# Autodesk Inventor assembly: Antriebsstrang
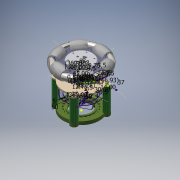
[picture p0: Inventor's stored thumbnail of the model, 180x180]
Saved by Autodesk Inventor 2018.3 (Build 223284000, 284)
## iProperties
Created: 2018-06-25
Part Number: Antriebsstrang
Material: Generisch
Document SubType Name: Assembly
Designer: JochenAlt
Author: JochenAlt
## Documents named in this file (5)
- D:\Projects\FlowerPot\CAD\Antriebsstrang.iam
- D:\Projects\FlowerPot\CAD\OmniWheel.ipt
- D:\Projects\FlowerPot\CAD\HarmonicDrive.iam
- D:\Projects\FlowerPot\CAD\Mounting Hub.ipt
- C:\Users\JochenAlt\Documents\Inventor\Content Center Files\R2018\de-DE\SKF - Single row ball bearings\SKF604.ipt
## Components (4 placed, 4 different names)
1. OmniWheel:1 — Passend:1, Passend:6, Passend:7, Passend:8
2. HarmonicDrive:1 [sub-assembly] — Passend:2, Passend:4, Passend:5, Passend:6
3. Mounting Hub:1 — Passend:1, Passend:2, Passend:5, Passend:7, Passend:8, Passend:9
4. SKF- Kugellager, einreihig SKF604:1 — Passend:4, Passend:9
## Relationships (8: Mate 8)
- Passend:1 [Mate]: OmniWheel:1 ↔ Mounting Hub:1
- Passend:2 [Mate]: HarmonicDrive:1 ↔ Mounting Hub:1
- Passend:4 [Mate]: HarmonicDrive:1 ↔ SKF- Kugellager, einreihig SKF604:1
- Passend:5 [Mate]: HarmonicDrive:1 ↔ Mounting Hub:1
- Passend:6 [Mate]: OmniWheel:1 ↔ HarmonicDrive:1
- Passend:7 [Mate]: OmniWheel:1 ↔ Mounting Hub:1
- Passend:8 [Mate]: OmniWheel:1 ↔ Mounting Hub:1
- Passend:9 [Mate] (0.5 mm): Mounting Hub:1 ↔ SKF- Kugellager, einreihig SKF604:1
